# Autodesk Inventor assembly: Type 1A 總組合 組合1
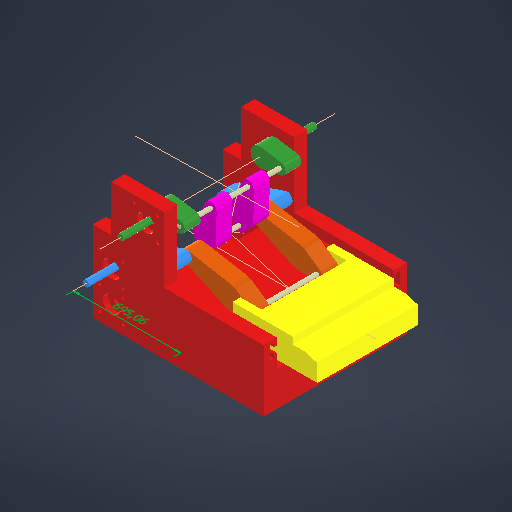
[picture p0: Inventor's stored thumbnail of the model, 512x512]
Saved by Autodesk Inventor 2025.3 (Build 293356030, 356C)
## iProperties
RuleStatus: InUse
Created: 2024-09-21
Part Number: Type 1A 總組合 組合1
Document SubType Name: Assembly
Designer: veter
Mass: 2.9492e+06 g
Surface Area: 86175 cm^2
Volume: 375694 cm^3
Density: 7.84999 g/cm^3
Author: veter
## Documents named in this file (8)
- C:\Users\Ou918\Downloads\AI-optimization\reference\model\Type 1A 總組合 組合1.iam
- C:\Users\Ou918\Downloads\AI-optimization\reference\model\Type 1A R1前充座.ipt
- C:\Users\Ou918\Downloads\AI-optimization\reference\model\Type 1A R2延伸曲柄.ipt
- C:\Users\Ou918\Downloads\AI-optimization\reference\model\Type 1A R3延伸連接桿.ipt
- C:\Users\Ou918\Downloads\AI-optimization\reference\model\Type 1A R4主滑台曲柄.ipt
- C:\Users\Ou918\Downloads\AI-optimization\reference\model\Type 1A R5主滑台連接桿.ipt
- C:\Users\Ou918\Downloads\AI-optimization\reference\model\Type 1A R6主滑台.ipt
- C:\Users\Ou918\Downloads\AI-optimization\reference\model\Type 1A 連接軸 1.ipt
## Components (9 placed, 7 different names)
1. Type 1A R1前充座:1 — J12, J14, J16
2. Type 1A R2延伸曲柄:1 — J12, 剛性:1, J23, 角度:1
3. Type 1A R3延伸連接桿:1 — J34, J23, J35
4. Type 1A R4主滑台曲柄:1 — J14, 剛性:2, J34, J45
5. Type 1A R5主滑台連接桿:1 — J35, J45, J56
6. Type 1A R6主滑台:1 — J16, J56, 剛性:3
7. Type 1A 連接軸 1:7 — 剛性:1
8. Type 1A 連接軸 1:8 — 剛性:2
9. Type 1A 連接軸 1:9 — 剛性:3
## Relationships (12: RevoluteJoint 5, WeldJoint 3, CylindricalJoint 2, TranslationJoint 1, Angle 1)
- J12 [RevoluteJoint]: Type 1A R1前充座:1 ↔ Type 1A R2延伸曲柄:1
- J14 [RevoluteJoint]: Type 1A R1前充座:1 ↔ Type 1A R4主滑台曲柄:1
- J16 [TranslationJoint]: Type 1A R1前充座:1 ↔ Type 1A R6主滑台:1
- J23 [CylindricalJoint]: Type 1A R2延伸曲柄:1 ↔ Type 1A R3延伸連接桿:1
- J34 [RevoluteJoint] (-103 mm): Type 1A R3延伸連接桿:1 ↔ Type 1A R4主滑台曲柄:1
- J35 [CylindricalJoint]: Type 1A R3延伸連接桿:1 ↔ Type 1A R5主滑台連接桿:1
- J45 [RevoluteJoint]: Type 1A R4主滑台曲柄:1 ↔ Type 1A R5主滑台連接桿:1
- J56 [RevoluteJoint]: Type 1A R5主滑台連接桿:1 ↔ Type 1A R6主滑台:1
- 剛性:1 [WeldJoint]: Type 1A R2延伸曲柄:1 ↔ Type 1A 連接軸 1:7
- 剛性:2 [WeldJoint]: Type 1A R4主滑台曲柄:1 ↔ Type 1A 連接軸 1:8
- 剛性:3 [WeldJoint]: Type 1A R6主滑台:1 ↔ Type 1A 連接軸 1:9
- 角度:1 [Angle] (89 deg): Type 1A R2延伸曲柄:1
## Named parameters: con_th = 45 deg
